# Autodesk Inventor assembly: RoadBot Pneumatic Module - with Jack - full assembly - r3
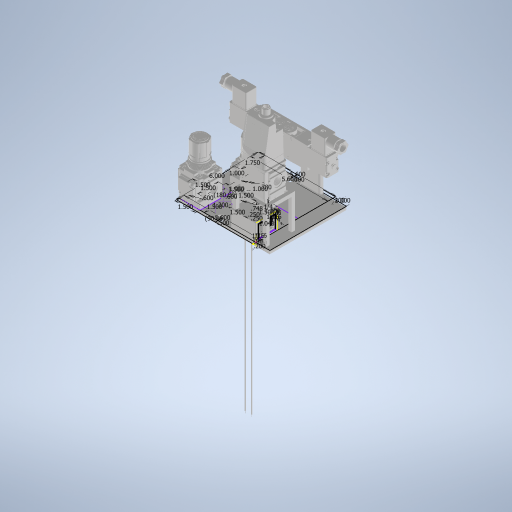
[picture p0: Inventor's stored thumbnail of the model, 512x512]
Saved by Autodesk Inventor 2024.1 (Build 281209000, 209)
## iProperties
Created: 2022-04-02
Part Number: RoadBot Pneumatic Module - with Jack - full assembly - r3
Document SubType Name: Assembly
Designer: Beaucage
Author: Beaucage
## Documents named in this file (7)
- C:\Users\pab2\Documents\GitHub\AFL-hardware-devel\AFL-Platform\LoaderGen2\TravelRobotFormFactor\RoadBot Pneumatic Module - with Jack - full assembly - r3.iam
- C:\Users\pab2\Documents\GitHub\AFL-hardware-devel\AFL-Platform\LoaderGen2\TravelRobotFormFactor\Keystone_Jack_Single_Receptacle (1).ipt
- C:\Users\pab2\Documents\GitHub\AFL-hardware-devel\AFL-Platform\LoaderGen2\TravelRobotFormFactor\RoadBot Pneumatic Module - Base - r3.ipt
- C:\Users\pab2\Downloads\8812K52_Compressed Air Regulator\8812K52_Compressed Air Regulator.ipt
- C:\Users\pab2\Downloads\5001T36_Miniature Solenoid On-Off Valve\5001T36_Miniature Solenoid On-Off Valve.ipt
- C:\Users\pab2\Downloads\8083T1_Precision Compressed Air Regulator with Display\8083T1_Precision Compressed Air Regulator with Display.ipt
- C:\Users\pab2\Downloads\6425K183_Electrical Air Directional Control Valve\6425K183_Electrical Air Directional Control Valve.ipt
## Components (7 placed, 6 different names)
1. RoadBot Pneumatic Module - Base - r3:1 — Mate:1, Mate:2, Flush:1, Mate:3, Mate:4, Mate:5, Mate:6, Mate:7, Mate:8, Mate:9, Mate:10, Mate:11, Mate:12
2. Keystone_Jack_Single_Receptacle (1):1 — Mate:1, Mate:2, Flush:1
3. 8812K52_Compressed Air Regulator:1 — Mate:3, Mate:7
4. 8812K52_Compressed Air Regulator:2 — Mate:4, Mate:8
5. 5001T36_Miniature Solenoid On-Off Valve:1 — Mate:5, Mate:6
6. 8083T1_Precision Compressed Air Regulator with Display:1 — Mate:9
7. 6425K183_Electrical Air Directional Control Valve:1 — Mate:10, Mate:11, Mate:12
## Relationships (13: Mate 12, Flush 1)
- Mate:1: RoadBot Pneumatic Module - Base - r3:1 ↔ Keystone_Jack_Single_Receptacle (1):1
- Mate:2: RoadBot Pneumatic Module - Base - r3:1 ↔ Keystone_Jack_Single_Receptacle (1):1
- Flush:1: RoadBot Pneumatic Module - Base - r3:1 ↔ Keystone_Jack_Single_Receptacle (1):1
- Mate:3: RoadBot Pneumatic Module - Base - r3:1 ↔ 8812K52_Compressed Air Regulator:1
- Mate:4: RoadBot Pneumatic Module - Base - r3:1 ↔ 8812K52_Compressed Air Regulator:2
- Mate:5: RoadBot Pneumatic Module - Base - r3:1 ↔ 5001T36_Miniature Solenoid On-Off Valve:1
- Mate:6 (6.35 mm): RoadBot Pneumatic Module - Base - r3:1 ↔ 5001T36_Miniature Solenoid On-Off Valve:1
- Mate:7: RoadBot Pneumatic Module - Base - r3:1 ↔ 8812K52_Compressed Air Regulator:1
- Mate:8: RoadBot Pneumatic Module - Base - r3:1 ↔ 8812K52_Compressed Air Regulator:2
- Mate:9: RoadBot Pneumatic Module - Base - r3:1 ↔ 8083T1_Precision Compressed Air Regulator with Display:1
- Mate:10: RoadBot Pneumatic Module - Base - r3:1 ↔ 6425K183_Electrical Air Directional Control Valve:1
- Mate:11: RoadBot Pneumatic Module - Base - r3:1 ↔ 6425K183_Electrical Air Directional Control Valve:1
- Mate:12: RoadBot Pneumatic Module - Base - r3:1 ↔ 6425K183_Electrical Air Directional Control Valve:1
